# Autodesk Inventor assembly: DesignRootModel^PCB_ESP32-C3-MINI-1_V1(2)_PCB_ESP32-C3-MINI-1_V1
(part 3 of 3)
275. 355
276. 356
277. 357
278. 358
279. 359
280. 360
281. 361
282. 362
283. 363
284. 364
285. 365
286. 366
287. 367
288. 368
289. 369
290. 370
291. 371
292. 372
293. 373
294. 374
295. 375
296. 376
297. 377
298. 378
299. 379
300. 380
301. 381
302. 382
303. 383
304. 384
305. 385
306. 386
307. 387
308. 388
309. 389
310. 390
311. 391
312. 392
313. 393
314. 394
315. 395
316. 396
317. 397
318. 398
319. 399
320. 400
321. 401
322. 402
323. 403
324. 404
325. 405
326. 406
327. 407
328. 408
329. 409
330. 410
331. 411
332. 412
